# Autodesk Inventor assembly: launcher_assembly
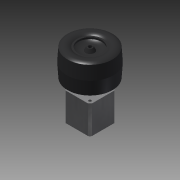
[picture p0: Inventor's stored thumbnail of the model, 180x180]
Saved by Autodesk Inventor 2013 (Build 170138000, 138)
## iProperties
Created: 2013-07-24
Part Number: launcher_assembly
Document SubType Name: Assembly
Designer: dkboone
Author: dkboone
## Documents named in this file (3)
- J:\groups\theresistors\Inventor\launcher_assembly.iam
- J:\groups\theresistors\Inventor\launcher_motor.ipt
- J:\groups\theresistors\Inventor\launcher_wheel.ipt
## Components (2 placed, 2 different names)
1. launcher_motor:1 — Mate:1, Mate:2
2. launcher_wheel:1 — Mate:1, Mate:2
## Relationships (2: Mate 2)
- Mate:1: launcher_motor:1 ↔ launcher_wheel:1
- Mate:2 (1.5875 mm): launcher_motor:1 ↔ launcher_wheel:1
